# Autodesk Inventor assembly: Servo Housing Assembly
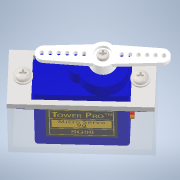
[picture p0: Inventor's stored thumbnail of the model, 180x180]
Saved by Autodesk Inventor 2022 (Build 260153000, 153)
## iProperties
Created: 2022-01-29
Part Number: Servo Housing Assembly
Document SubType Name: Assembly
Designer: peter
Author: peter
## Documents named in this file (5)
- C:\Users\peter\OneDrive\Desktop\sg90-micro-servo-9g-tower-pro-1.snapshot.3\Servo\Servo Housing Assembly.iam
- C:\Users\peter\OneDrive\Desktop\sg90-micro-servo-9g-tower-pro-1.snapshot.3\Servo\servo housing template.ipt
- C:\Users\peter\OneDrive\Desktop\sg90-micro-servo-9g-tower-pro-1.snapshot.3\Servo\servo housing lid.ipt
- C:\Users\peter\OneDrive\Desktop\sg90-micro-servo-9g-tower-pro-1.snapshot.3\Servo\SG90 - Micro Servo 9g - Tower Pro.iam
- C:\Users\peter\OneDrive\Desktop\sg90-micro-servo-9g-tower-pro-1.snapshot.3\Servo\servo housing.ipt
## Components (4 placed, 4 different names)
1. servo housing:1 — Rigid:1
2. servo housing template:1 — Rigid:2
3. servo housing lid:1 — Rigid:1, Rigid:2, Rigid:3
4. SG90 - Micro Servo 9g - Tower Pro:1 [sub-assembly] — Rigid:3
## Relationships (3: WeldJoint 3)
- Rigid:1 [WeldJoint]: servo housing:1 ↔ servo housing lid:1
- Rigid:2 [WeldJoint] (2.5 mm): servo housing template:1 ↔ servo housing lid:1
- Rigid:3 [WeldJoint] (2.5 mm): servo housing lid:1 ↔ SG90 - Micro Servo 9g - Tower Pro:1
